# Autodesk Inventor assembly: Kit Frame 26x30
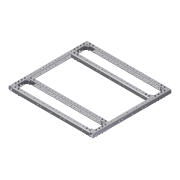
[picture p0: Inventor's stored thumbnail of the model, 180x180]
Saved by Autodesk Inventor 2013 (Build 170138000, 138)
## iProperties
Created: 2013-01-06
Part Number: Kit Frame 26x30
Document SubType Name: Assembly
Designer: Nemo
Author: Nemo
## Documents named in this file (4)
- H:\Nemo\Documents\Robotics\COTS Parts\Kit Frame\Kit Frame 28x28.iam
- H:\Nemo\Documents\Robotics\COTS Parts\Kit Frame\Components\C Channel - FrontBack 26x30.ipt
- H:\Nemo\Documents\Robotics\COTS Parts\Kit Frame\Components\28x28 Side Rail sub.iam
- H:\Nemo\Documents\Robotics\COTS Parts\Kit Frame\Components\28x28 Side Rail Sub mirror.iam
## Components (6 placed, 3 different names)
1. C Channel - Cut-01:3 — Flush:5, Flush:6, Mate:6
2. C Channel - Cut-01:4 — Mate:3, Mate:4, Flush:6, Insert:1, Mate:5, Insert:2, Mate:7, Insert:3, Mate:8, Insert:4, Mate:9
3. 28x28 Side Rail sub:1 [sub-assembly] — Insert:1, Mate:5, Mate:6, Flush:7
4. 28x28 Side Rail Sub mirror:1 [sub-assembly] — Insert:2, Mate:7
5. 28x28 Side Rail sub:2 [sub-assembly] — Insert:4, Mate:9
6. 28x28 Side Rail Sub mirror:2 [sub-assembly] — Insert:3, Mate:8
## Relationships (14: Mate 7, Insert 4, Flush 3)
- Flush:5: C Channel - Cut-01:3
- Mate:3: C Channel - Cut-01:4
- Mate:4 (36.83 mm): C Channel - Cut-01:4
- Flush:6: C Channel - Cut-01:3 ↔ C Channel - Cut-01:4
- Insert:1: C Channel - Cut-01:4 ↔ 28x28 Side Rail sub:1
- Mate:5: C Channel - Cut-01:4 ↔ 28x28 Side Rail sub:1
- Mate:6: C Channel - Cut-01:3 ↔ 28x28 Side Rail sub:1
- Flush:7: 28x28 Side Rail sub:1
- Insert:2: C Channel - Cut-01:4 ↔ 28x28 Side Rail Sub mirror:1
- Mate:7: C Channel - Cut-01:4 ↔ 28x28 Side Rail Sub mirror:1
- Insert:3: C Channel - Cut-01:4 ↔ 28x28 Side Rail Sub mirror:2
- Mate:8: C Channel - Cut-01:4 ↔ 28x28 Side Rail Sub mirror:2
- Insert:4: C Channel - Cut-01:4 ↔ 28x28 Side Rail sub:2
- Mate:9: C Channel - Cut-01:4 ↔ 28x28 Side Rail sub:2
